# Autodesk Inventor assembly: scara
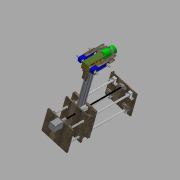
[picture p0: Inventor's stored thumbnail of the model, 180x180]
Saved by Autodesk Inventor 2019 (Build 230136000, 136)
## iProperties
Created: 2021-11-05
Part Number: scara
Document SubType Name: Assembly
Designer: Mohamed
Author: Mohamed
## Documents named in this file (4)
- F:\Semester 7\Design of mechatronics 1\SSCARA Robot\scara.iam
- F:\Semester 7\Design of mechatronics 1\SSCARA Robot\elevator.iam
- F:\Semester 7\Design of mechatronics 1\SSCARA Robot\Griper_v slot.iam
- F:\Semester 7\Design of mechatronics 1\SSCARA Robot\Tower.iam
## Components (3 placed, 3 different names)
1. elevator:1 [sub-assembly] — Mate:1, Mate:2, Mate:3, Mate:4, Mate:5
2. Griper_v slot:1 [sub-assembly] — Mate:1, Mate:2, Mate:3
3. Tower:1 [sub-assembly] — Mate:4, Mate:5
## Relationships (5: Mate 5)
- Mate:1: elevator:1 ↔ Griper_v slot:1
- Mate:2: elevator:1 ↔ Griper_v slot:1
- Mate:3: elevator:1 ↔ Griper_v slot:1
- Mate:4: elevator:1 ↔ Tower:1
- Mate:5: elevator:1 ↔ Tower:1
